(part 1 of 3)
# Autodesk Inventor assembly: 42146-00
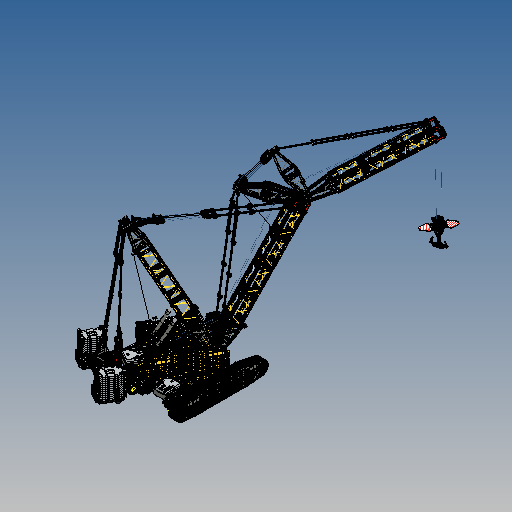
[picture p0: Inventor's stored thumbnail of the model, 512x512]
Saved by Autodesk Inventor 2025 (Build 290162010, 162A)
## iProperties
Created: 2024-11-13
Part Number: 42146-00
Material: Generisch
Document SubType Name: Assembly
Designer: hp.muther
Author: hp.muther
## Documents named in this file (138)
- D:\Inventor\Projekte\LEGO Technik - Raupenkran LR 13000 (42146)\LEGO Technik - Raupenkran LR 13000 (42146).iam
- D:\Inventor\Projekte\LEGO Technik - Raupenkran LR 13000 (42146)\LEGO Technik - Raupenkran LR 13000 (42146)\42146-01.iam
- D:\Inventor\Projekte\LEGO Technik - Raupenkran LR 13000 (42146)\LEGO Technik - Raupenkran LR 13000 (42146)\42146-02.iam
- D:\Inventor\Projekte\LEGO Technik - Raupenkran LR 13000 (42146)\LEGO Technik - Raupenkran LR 13000 (42146)\42146-03.iam
- D:\Inventor\Projekte\LEGO Technik - Raupenkran LR 13000 (42146)\LEGO Pieces\32054-LtBluishGray.ipt
- D:\Inventor\Projekte\LEGO Technik - Raupenkran LR 13000 (42146)\LEGO Pieces\43093-Blue.ipt
- D:\Inventor\Projekte\LEGO Technik - Raupenkran LR 13000 (42146)\LEGO Technik - Raupenkran LR 13000 (42146)\42146-04.iam
- D:\Inventor\Projekte\LEGO Technik - Raupenkran LR 13000 (42146)\LEGO Technik - Raupenkran LR 13000 (42146)\42146-05.iam
- D:\Inventor\Projekte\LEGO Technik - Raupenkran LR 13000 (42146)\LEGO Pieces\6558-Blue.ipt
- D:\Inventor\Projekte\LEGO Technik - Raupenkran LR 13000 (42146)\LEGO Pieces\11214-Red.ipt
- D:\Inventor\Projekte\LEGO Technik - Raupenkran LR 13000 (42146)\LEGO Pieces\73507-Black.ipt
- D:\Inventor\Projekte\LEGO Technik - Raupenkran LR 13000 (42146)\LEGO Pieces\32524-Yellow.ipt
- D:\Inventor\Projekte\LEGO Technik - Raupenkran LR 13000 (42146)\LEGO Technik - Raupenkran LR 13000 (42146)\42146-06.iam
- D:\Inventor\Projekte\LEGO Technik - Raupenkran LR 13000 (42146)\LEGO Technik - Raupenkran LR 13000 (42146)\42146-07.iam
- D:\Inventor\Projekte\LEGO Technik - Raupenkran LR 13000 (42146)\LEGO Technik - Raupenkran LR 13000 (42146)\42146-08.iam
- D:\Inventor\Projekte\LEGO Technik - Raupenkran LR 13000 (42146)\LEGO Pieces\32278-Yellow.ipt
- D:\Inventor\Projekte\LEGO Technik - Raupenkran LR 13000 (42146)\LEGO Pieces\32525-Red.ipt
- D:\Inventor\Projekte\LEGO Technik - Raupenkran LR 13000 (42146)\LEGO Pieces\2780-Black.ipt
- D:\Inventor\Projekte\LEGO Technik - Raupenkran LR 13000 (42146)\LEGO Pieces\24316-ReddishBrown.ipt
- D:\Inventor\Projekte\LEGO Technik - Raupenkran LR 13000 (42146)\LEGO Pieces\46372-LtBluishGray.ipt
- D:\Inventor\Projekte\LEGO Technik - Raupenkran LR 13000 (42146)\LEGO Pieces\15458-DkBluishGray.ipt
- D:\Inventor\Projekte\LEGO Technik - Raupenkran LR 13000 (42146)\LEGO Pieces\67491-Yellow.ipt
- D:\Inventor\Projekte\LEGO Technik - Raupenkran LR 13000 (42146)\LEGO Pieces\40490-LtBluishGray.ipt
- D:\Inventor\Projekte\LEGO Technik - Raupenkran LR 13000 (42146)\LEGO Pieces\39790-Black.ipt
- D:\Inventor\Projekte\LEGO Technik - Raupenkran LR 13000 (42146)\LEGO Pieces\18651-Black.ipt
- D:\Inventor\Projekte\LEGO Technik - Raupenkran LR 13000 (42146)\LEGO Pieces\18654-DkBluishGray.ipt
- D:\Inventor\Projekte\LEGO Technik - Raupenkran LR 13000 (42146)\LEGO Technik - Raupenkran LR 13000 (42146)\42146-09.iam
- D:\Inventor\Projekte\LEGO Technik - Raupenkran LR 13000 (42146)\LEGO Pieces\32140-LtBluishGray.ipt
- D:\Inventor\Projekte\LEGO Technik - Raupenkran LR 13000 (42146)\LEGO Technik - Raupenkran LR 13000 (42146)\42146-10.iam
- D:\Inventor\Projekte\LEGO Technik - Raupenkran LR 13000 (42146)\LEGO Pieces\32278-LtBluishGray.ipt
- D:\Inventor\Projekte\LEGO Technik - Raupenkran LR 13000 (42146)\LEGO Pieces\43857-LtBluishGray.ipt
- D:\Inventor\Projekte\LEGO Technik - Raupenkran LR 13000 (42146)\LEGO Technik - Raupenkran LR 13000 (42146)\42146-11.iam
- D:\Inventor\Projekte\LEGO Technik - Raupenkran LR 13000 (42146)\LEGO Technik - Raupenkran LR 13000 (42146)\42146-12.iam
- D:\Inventor\Projekte\LEGO Technik - Raupenkran LR 13000 (42146)\LEGO Pieces\6629-DkBluishGray.ipt
- D:\Inventor\Projekte\LEGO Technik - Raupenkran LR 13000 (42146)\LEGO Technik - Raupenkran LR 13000 (42146)\42146-13.iam
- D:\Inventor\Projekte\LEGO Technik - Raupenkran LR 13000 (42146)\LEGO Technik - Raupenkran LR 13000 (42146)\42146-14.iam
- D:\Inventor\Projekte\LEGO Technik - Raupenkran LR 13000 (42146)\LEGO Pieces\6589-Tan.ipt
- D:\Inventor\Projekte\LEGO Technik - Raupenkran LR 13000 (42146)\LEGO Pieces\62462-LtBluishGray.ipt
- D:\Inventor\Projekte\LEGO Technik - Raupenkran LR 13000 (42146)\LEGO Pieces\15462-ReddishBrown.ipt
- D:\Inventor\Projekte\LEGO Technik - Raupenkran LR 13000 (42146)\LEGO Pieces\32316-LtBluishGray.ipt
- D:\Inventor\Projekte\LEGO Technik - Raupenkran LR 13000 (42146)\LEGO Pieces\18945-DkBluishGray.ipt
- D:\Inventor\Projekte\LEGO Technik - Raupenkran LR 13000 (42146)\LEGO Pieces\60483-DkBluishGray.ipt
- D:\Inventor\Projekte\LEGO Technik - Raupenkran LR 13000 (42146)\LEGO Pieces\32316-DkBluishGray.ipt
- D:\Inventor\Projekte\LEGO Technik - Raupenkran LR 13000 (42146)\LEGO Pieces\771710-DkBluishGray.ipt
- D:\Inventor\Projekte\LEGO Technik - Raupenkran LR 13000 (42146)\LEGO Pieces\11947-DkBluishGray.ipt
- D:\Inventor\Projekte\LEGO Technik - Raupenkran LR 13000 (42146)\LEGO Pieces\3713-LtBluishGray.ipt
- D:\Inventor\Projekte\LEGO Technik - Raupenkran LR 13000 (42146)\LEGO Technik - Raupenkran LR 13000 (42146)\42146-15.iam
- D:\Inventor\Projekte\LEGO Technik - Raupenkran LR 13000 (42146)\LEGO Pieces\11946-DkBluishGray.ipt
- D:\Inventor\Projekte\LEGO Technik - Raupenkran LR 13000 (42146)\LEGO Technik - Raupenkran LR 13000 (42146)\42146-16.iam
- D:\Inventor\Projekte\LEGO Technik - Raupenkran LR 13000 (42146)\LEGO Technik - Raupenkran LR 13000 (42146)\42146-17.iam
- D:\Inventor\Projekte\LEGO Technik - Raupenkran LR 13000 (42146)\LEGO Pieces\40490-DkBluishGray.ipt
- D:\Inventor\Projekte\LEGO Technik - Raupenkran LR 13000 (42146)\LEGO Technik - Raupenkran LR 13000 (42146)\42146-18.iam
- D:\Inventor\Projekte\LEGO Technik - Raupenkran LR 13000 (42146)\LEGO Technik - Raupenkran LR 13000 (42146)\42146-19.iam
- D:\Inventor\Projekte\LEGO Technik - Raupenkran LR 13000 (42146)\LEGO Technik - Raupenkran LR 13000 (42146)\42146-20.iam
- D:\Inventor\Projekte\LEGO Technik - Raupenkran LR 13000 (42146)\LEGO Pieces\32526-Yellow.ipt
- D:\Inventor\Projekte\LEGO Technik - Raupenkran LR 13000 (42146)\LEGO Pieces\60484-Yellow.ipt
- D:\Inventor\Projekte\LEGO Technik - Raupenkran LR 13000 (42146)\LEGO Pieces\3673-LtBluishGray.ipt
- D:\Inventor\Projekte\LEGO Technik - Raupenkran LR 13000 (42146)\LEGO Technik - Raupenkran LR 13000 (42146)\42146-21.iam
- D:\Inventor\Projekte\LEGO Technik - Raupenkran LR 13000 (42146)\LEGO Pieces\771710-Black.ipt
- D:\Inventor\Projekte\LEGO Technik - Raupenkran LR 13000 (42146)\LEGO Pieces\32002-Tan.ipt
- D:\Inventor\Projekte\LEGO Technik - Raupenkran LR 13000 (42146)\LEGO Pieces\32525-Yellow.ipt
- D:\Inventor\Projekte\LEGO Technik - Raupenkran LR 13000 (42146)\LEGO Pieces\18942-DkBluishGray.ipt
- D:\Inventor\Projekte\LEGO Technik - Raupenkran LR 13000 (42146)\LEGO Pieces\18940-SandBlue.ipt
- D:\Inventor\Projekte\LEGO Technik - Raupenkran LR 13000 (42146)\LEGO Pieces\18654-Black.ipt
- D:\Inventor\Projekte\LEGO Technik - Raupenkran LR 13000 (42146)\LEGO Pieces\32073-LtBluishGray.ipt
- D:\Inventor\Projekte\LEGO Technik - Raupenkran LR 13000 (42146)\LEGO Pieces\60485-LtBluishGray.ipt
- D:\Inventor\Projekte\LEGO Technik - Raupenkran LR 13000 (42146)\LEGO Pieces\32184-LtBluishGray.ipt
- D:\Inventor\Projekte\LEGO Technik - Raupenkran LR 13000 (42146)\LEGO Pieces\77765-MediumStoneGrey.ipt
- D:\Inventor\Projekte\LEGO Technik - Raupenkran LR 13000 (42146)\LEGO Pieces\4265c-Yellow.ipt
- D:\Inventor\Projekte\LEGO Technik - Raupenkran LR 13000 (42146)\LEGO Pieces\32017-DKBluishGray.ipt
- D:\Inventor\Projekte\LEGO Technik - Raupenkran LR 13000 (42146)\LEGO Pieces\6628-Red.ipt
- D:\Inventor\Projekte\LEGO Technik - Raupenkran LR 13000 (42146)\LEGO Technik - Raupenkran LR 13000 (42146)\42146_70902_1.ipt
- D:\Inventor\Projekte\LEGO Technik - Raupenkran LR 13000 (42146)\LEGO Technik - Raupenkran LR 13000 (42146)\42146-22.iam
- D:\Inventor\Projekte\LEGO Technik - Raupenkran LR 13000 (42146)\LEGO Technik - Raupenkran LR 13000 (42146)\42146-23.iam
- D:\Inventor\Projekte\LEGO Technik - Raupenkran LR 13000 (42146)\LEGO Technik - Raupenkran LR 13000 (42146)\42146-24.iam
- D:\Inventor\Projekte\LEGO Technik - Raupenkran LR 13000 (42146)\LEGO Technik - Raupenkran LR 13000 (42146)\42146-25.iam
- D:\Inventor\Projekte\LEGO Technik - Raupenkran LR 13000 (42146)\LEGO Pieces\85824 - HUB.iam
- D:\Inventor\Projekte\LEGO Technik - Raupenkran LR 13000 (42146)\LEGO Pieces\84428-LtBluishGray.ipt
- D:\Inventor\Projekte\LEGO Technik - Raupenkran LR 13000 (42146)\LEGO Pieces\79768-DkBluishGray.ipt
- D:\Inventor\Projekte\LEGO Technik - Raupenkran LR 13000 (42146)\LEGO Pieces\6536-Yellow.ipt
- D:\Inventor\Projekte\LEGO Technik - Raupenkran LR 13000 (42146)\LEGO Pieces\32525-LtBluishGray.ipt
- D:\Inventor\Projekte\LEGO Technik - Raupenkran LR 13000 (42146)\LEGO Technik - Raupenkran LR 13000 (42146)\42146-26.iam
- D:\Inventor\Projekte\LEGO Technik - Raupenkran LR 13000 (42146)\LEGO Pieces\67498-shock absorber.iam
- D:\Inventor\Projekte\LEGO Technik - Raupenkran LR 13000 (42146)\LEGO Technik - Raupenkran LR 13000 (42146)\42146-27.iam
- D:\Inventor\Projekte\LEGO Technik - Raupenkran LR 13000 (42146)\LEGO Pieces\44294-Yellow.ipt
- D:\Inventor\Projekte\LEGO Technik - Raupenkran LR 13000 (42146)\LEGO Pieces\2637-LtBluishGray.ipt
- D:\Inventor\Projekte\LEGO Technik - Raupenkran LR 13000 (42146)\LEGO Pieces\6632-LtBluishGray.ipt
- D:\Inventor\Projekte\LEGO Technik - Raupenkran LR 13000 (42146)\LEGO Pieces\32449-Yellow.ipt
- D:\Inventor\Projekte\LEGO Technik - Raupenkran LR 13000 (42146)\LEGO Pieces\32062-Red.ipt
- D:\Inventor\Projekte\LEGO Technik - Raupenkran LR 13000 (42146)\LEGO Pieces\4519-Yellow.ipt
- D:\Inventor\Projekte\LEGO Technik - Raupenkran LR 13000 (42146)\LEGO Pieces\3707-Black.ipt
- D:\Inventor\Projekte\LEGO Technik - Raupenkran LR 13000 (42146)\LEGO Pieces\32184-Yellow.ipt
- D:\Inventor\Projekte\LEGO Technik - Raupenkran LR 13000 (42146)\LEGO Pieces\48989-LtBluishGray.ipt
- D:\Inventor\Projekte\LEGO Technik - Raupenkran LR 13000 (42146)\LEGO Pieces\32524-LtBluishGray.ipt
- D:\Inventor\Projekte\LEGO Technik - Raupenkran LR 13000 (42146)\LEGO Pieces\40490-Yellow.ipt
- D:\Inventor\Projekte\LEGO Technik - Raupenkran LR 13000 (42146)\LEGO Pieces\18939-LIGHTGREY.ipt
- D:\Inventor\Projekte\LEGO Technik - Raupenkran LR 13000 (42146)\LEGO Technik - Raupenkran LR 13000 (42146)\42146-28.iam
- D:\Inventor\Projekte\LEGO Technik - Raupenkran LR 13000 (42146)\LEGO Technik - Raupenkran LR 13000 (42146)\42146-29.iam
- D:\Inventor\Projekte\LEGO Technik - Raupenkran LR 13000 (42146)\LEGO Pieces\41677-LtBluishGray.ipt
- D:\Inventor\Projekte\LEGO Technik - Raupenkran LR 13000 (42146)\LEGO Pieces\6538c-Red.ipt
- D:\Inventor\Projekte\LEGO Technik - Raupenkran LR 13000 (42146)\LEGO Pieces\11478-LtBluishGray.ipt
- D:\Inventor\Projekte\LEGO Technik - Raupenkran LR 13000 (42146)\LEGO Pieces\42610-LtBluishGray.ipt
- D:\Inventor\Projekte\LEGO Technik - Raupenkran LR 13000 (42146)\LEGO Pieces\26287-LtBluishGray.ipt
- D:\Inventor\Projekte\LEGO Technik - Raupenkran LR 13000 (42146)\LEGO Pieces\92907-LtBluishGray.ipt
- D:\Inventor\Projekte\LEGO Technik - Raupenkran LR 13000 (42146)\LEGO Pieces\80295-White.ipt
- D:\Inventor\Projekte\LEGO Technik - Raupenkran LR 13000 (42146)\LEGO Pieces\23948-Yellow.ipt
- D:\Inventor\Projekte\LEGO Technik - Raupenkran LR 13000 (42146)\LEGO Technik - Raupenkran LR 13000 (42146)\42146-30.iam
- D:\Inventor\Projekte\LEGO Technik - Raupenkran LR 13000 (42146)\LEGO Pieces\4274-Red.ipt
- D:\Inventor\Projekte\LEGO Technik - Raupenkran LR 13000 (42146)\LEGO Pieces\64179-Red.ipt
- D:\Inventor\Projekte\LEGO Technik - Raupenkran LR 13000 (42146)\LEGO Pieces\58176-TransRed.ipt
- D:\Inventor\Projekte\LEGO Technik - Raupenkran LR 13000 (42146)\LEGO Technik - Raupenkran LR 13000 (42146)\42146-31.iam
- D:\Inventor\Projekte\LEGO Technik - Raupenkran LR 13000 (42146)\LEGO Pieces\3706-Red.ipt
- D:\Inventor\Projekte\LEGO Technik - Raupenkran LR 13000 (42146)\LEGO Technik - Raupenkran LR 13000 (42146)\42146-32.iam
- D:\Inventor\Projekte\LEGO Technik - Raupenkran LR 13000 (42146)\LEGO Pieces\62462-Yellow.ipt
- D:\Inventor\Projekte\LEGO Technik - Raupenkran LR 13000 (42146)\LEGO Technik - Raupenkran LR 13000 (42146)\42146-33.iam
- D:\Inventor\Projekte\LEGO Technik - Raupenkran LR 13000 (42146)\LEGO Technik - Raupenkran LR 13000 (42146)\42146-34.iam
- D:\Inventor\Projekte\LEGO Technik - Raupenkran LR 13000 (42146)\LEGO Technik - Raupenkran LR 13000 (42146)\42146-35.iam
- D:\Inventor\Projekte\LEGO Technik - Raupenkran LR 13000 (42146)\LEGO Pieces\4519-LtBluishGray.ipt
- D:\Inventor\Projekte\LEGO Technik - Raupenkran LR 13000 (42146)\LEGO Pieces\41677-DKBluishGray.ipt
- D:\Inventor\Projekte\LEGO Technik - Raupenkran LR 13000 (42146)\LEGO Pieces\25214-LtBluishGray.ipt
- D:\Inventor\Projekte\LEGO Technik - Raupenkran LR 13000 (42146)\LEGO Technik - Raupenkran LR 13000 (42146)\42146-36.iam
- D:\Inventor\Projekte\LEGO Technik - Raupenkran LR 13000 (42146)\LEGO Pieces\4162-LtBluishGray.ipt
- D:\Inventor\Projekte\LEGO Technik - Raupenkran LR 13000 (42146)\LEGO Pieces\3022-Yellow.ipt
- D:\Inventor\Projekte\LEGO Technik - Raupenkran LR 13000 (42146)\LEGO Pieces\3710-Yellow.ipt
- D:\Inventor\Projekte\LEGO Technik - Raupenkran LR 13000 (42146)\LEGO Pieces\2420-Yellow.ipt
- D:\Inventor\Projekte\LEGO Technik - Raupenkran LR 13000 (42146)\LEGO Pieces\3020-Yellow.ipt
- D:\Inventor\Projekte\LEGO Technik - Raupenkran LR 13000 (42146)\LEGO Pieces\44873-LtBluishGray.ipt
- D:\Inventor\Projekte\LEGO Technik - Raupenkran LR 13000 (42146)\LEGO Pieces\87994-LtBluishGray.ipt
- D:\Inventor\Projekte\LEGO Technik - Raupenkran LR 13000 (42146)\LEGO Pieces\63037-LtBluishGray.ipt
- D:\Inventor\Projekte\LEGO Technik - Raupenkran LR 13000 (42146)\LEGO Pieces\63965-LtBluishGray.ipt
- D:\Inventor\Projekte\LEGO Technik - Raupenkran LR 13000 (42146)\LEGO Pieces\4274-LtBluishGray.ipt
- D:\Inventor\Projekte\LEGO Technik - Raupenkran LR 13000 (42146)\LEGO Pieces\3023-Black.ipt
- D:\Inventor\Projekte\LEGO Technik - Raupenkran LR 13000 (42146)\LEGO Pieces\54200-TransClear.ipt
- D:\Inventor\Projekte\LEGO Technik - Raupenkran LR 13000 (42146)\LEGO Pieces\32291-DkBluishGray.ipt
- D:\Inventor\Projekte\LEGO Technik - Raupenkran LR 13000 (42146)\LEGO Technik - Raupenkran LR 13000 (42146)\42146-37.iam
- D:\Inventor\Projekte\LEGO Technik - Raupenkran LR 13000 (42146)\LEGO Technik - Raupenkran LR 13000 (42146)\42146-38.ipt
- D:\Inventor\Projekte\LEGO Technik - Raupenkran LR 13000 (42146)\LEGO Technik - Raupenkran LR 13000 (42146)\42146-39.ipt
- D:\Inventor\Projekte\LEGO Technik - Raupenkran LR 13000 (42146)\LEGO Technik - Raupenkran LR 13000 (42146)\42146-40.ipt
## Components (648 placed, 137 different names)
1. 42146-38:1 — Passend:501, Passend:502, Winkel:20
2. 80295-White:1 — Einfügen:488
3. 23948-Yellow:1 — Einfügen:487, Einfügen:488, Passend:502
4. 42146-39:1 — Passend:503, Passend:504, Winkel:21
5. 80295-White:2 — Einfügen:536
6. 23948-Yellow:2 — Passend:504
7. 42146-40:1 — Passend:505, Passend:506, Winkel:22
8. 80295-White:3 — Einfügen:577
9. 80295-White:4 — Einfügen:576, Einfügen:577
10. 23948-Yellow:3 — Einfügen:576, Einfügen:578, Passend:506
11. 42146-01:1 [sub-assembly] — Passend:1, Passend:2, Passend:3, Fluchtend:1, Einfügen:1, Passend:4, Einfügen:2, Passend:5, Einfügen:5, Einfügen:6, Passend:10, Passend:11, Passend:12, Einfügen:15, Einfügen:16, Einfügen:17, Einfügen:18, Passend:13, Einfügen:20, Einfügen:21, Einfügen:22, Einfügen:23, Einfügen:24, Einfügen:25, Einfügen:26, Einfügen:27, Einfügen:28
12. 42146-02:1 [sub-assembly] — Einfügen:1, Passend:4, Einfügen:4, Einfügen:7, Einfügen:8, Einfügen:71, Passend:42, Einfügen:74
13. 42146-03:1 [sub-assembly] — Einfügen:2, Passend:5, Einfügen:3, Passend:6, Passend:7, Einfügen:72, Passend:41, Winkel:19
14. 42146-04:1 [sub-assembly] — Einfügen:7, Passend:6
15. 42146-05:1 [sub-assembly] — Einfügen:8, Passend:7, Passend:14, Einfügen:19
16. 42146-06:1 [sub-assembly] — Passend:13, Passend:14
17. 42146-07:1 [sub-assembly] — Einfügen:19, Passend:32, Passend:34, Einfügen:33, Passend:36, Passend:17, Passend:18, Passend:19, Passend:20, Drehung:1, Drehung:2, Passend:25, Passend:33, Passend:35, Passend:37, Passend:38
18. 42146-08:1 - beweglich [sub-assembly] — Einfügen:28, Passend:15, Einfügen:45, Passend:22, Einfügen:46, Passend:23, Einfügen:47
19. 42146-09:1 [sub-assembly] — Einfügen:76, Passend:43, Einfügen:80, Passend:44, Einfügen:86, Einfügen:87, Passend:49, Einfügen:94, Einfügen:96, Einfügen:98, Einfügen:100, Einfügen:101, Einfügen:106, Passend:52, Einfügen:121, Passend:59, Einfügen:130, Einfügen:146, Passend:67, Einfügen:181, Passend:82, Einfügen:183, Passend:84, Einfügen:195, Einfügen:196, Einfügen:197, Einfügen:198, Einfügen:207, Einfügen:208
20. 42146-10:1 [sub-assembly] — Einfügen:81, Passend:45, Einfügen:85, Passend:46, Passend:47, Einfügen:88, Einfügen:92, Einfügen:93, Einfügen:95, Einfügen:97, Einfügen:99, Einfügen:113, Passend:56, Einfügen:151, Passend:71, Passend:80, Einfügen:180, Passend:81, Einfügen:182, Passend:83, Einfügen:184, Passend:85, Einfügen:199, Einfügen:200, Einfügen:201, Einfügen:202, Einfügen:205, Einfügen:206
21. 42146-11:1 [sub-assembly] — Einfügen:101, Passend:50, Einfügen:102, Einfügen:103, Einfügen:104, Einfügen:105
22. 42146-12:1 [sub-assembly] — Einfügen:106, Passend:52, Einfügen:111, Passend:54, Einfügen:112, Passend:55, Einfügen:192, Passend:89, Passend:93
23. 42146-13:1 [sub-assembly] — Einfügen:113, Passend:56, Einfügen:118, Passend:58, Einfügen:119, Einfügen:120, Einfügen:188, Passend:87, Passend:90, Passend:95
24. 42146-14:1 [sub-assembly] — Einfügen:121, Passend:59, Passend:61, Passend:68
25. 42146-15:1 [sub-assembly] — Einfügen:151, Passend:71, Einfügen:179, Einfügen:209, Passend:94
26. 42146-16:1 [sub-assembly] — Einfügen:182, Passend:83
27. 42146-16:2 [sub-assembly] — Einfügen:181, Passend:82
28. 42146-17:1 [sub-assembly] — Einfügen:183, Passend:84
29. 42146-17:2 [sub-assembly] — Einfügen:184, Passend:85
30. 42146-18:1 [sub-assembly] — Einfügen:209, Passend:94
31. 42146-19:1 [sub-assembly] — Passend:95, Passend:96, Winkel:1
32. 42146-19:2 [sub-assembly] — Passend:97, Winkel:2, Passend:98
33. 42146-20:1 [sub-assembly] — Einfügen:210, Passend:99, Einfügen:211, Einfügen:212, Einfügen:213, Einfügen:214, Einfügen:215, Einfügen:216, Einfügen:217, Einfügen:218, Einfügen:219, Einfügen:220, Einfügen:221, Einfügen:226, Einfügen:227, Einfügen:228, Einfügen:229, Einfügen:230, Einfügen:231, Einfügen:232, Einfügen:233, Einfügen:234, Einfügen:235, Einfügen:236, Einfügen:237, Einfügen:238, Einfügen:243, Einfügen:244, Einfügen:252, Passend:104, Einfügen:251, Passend:105, Einfügen:259, Einfügen:260, Passend:106, Passend:107, Einfügen:296, Einfügen:297, Einfügen:350, Passend:154, Einfügen:352, Einfügen:353, Einfügen:366, Einfügen:367, Einfügen:386, Einfügen:387, Einfügen:388, Einfügen:443, Einfügen:444, Einfügen:536, Passend:501, Winkel:20, Passend:503, Winkel:21, Passend:505, Winkel:22
34. 42146-21:1 [sub-assembly] — Einfügen:279, Passend:114, Passend:115, Passend:116, Passend:117, Passend:118, Einfügen:316, Passend:148, Passend:149
35. 42146-22:1 [sub-assembly] — Passend:145, Passend:146, Passend:147, Einfügen:381, Passend:239, Einfügen:382, Einfügen:383, Einfügen:384, Einfügen:385, Passend:240
36. 42146-23:1 [sub-assembly] — Einfügen:324, Passend:148, Passend:152, Passend:153, Passend:232, Passend:233, Passend:234
37. 42146-24:1 [sub-assembly] — Einfügen:323, Passend:149, Passend:150, Passend:151, Passend:163, Passend:164, Passend:165
38. 42146-25:1 [sub-assembly] — Einfügen:354, Passend:155, Passend:156, Passend:157, Einfügen:370, Passend:158, Einfügen:371, Passend:161, Einfügen:487, Einfügen:544, Passend:452, Einfügen:578
39. 42146-26:1 [sub-assembly] — Einfügen:388, Passend:243, Passend:244, Einfügen:395, Passend:245
40. 67498-shock absorber:1 [sub-assembly] — Einfügen:391, Einfügen:392, Einfügen:394, Passend:244
41. 67498-shock absorber:2 [sub-assembly] — Einfügen:389, Einfügen:390, Einfügen:393, Passend:243
42. 42146-27:1 [sub-assembly] — Einfügen:395, Passend:245, Einfügen:396, Einfügen:397, Einfügen:412, Passend:423, Fluchtend:14, Passend:435
43. 42146-28:1 [sub-assembly] — Einfügen:445, Passend:426, Einfügen:452, Passend:429, Einfügen:490, Passend:440, Passend:448, Einfügen:574, Einfügen:575, Passend:497
44. 42146-29:1 [sub-assembly] — Einfügen:452, Passend:429, Einfügen:485, Einfügen:486
45. 42146-30:1 [sub-assembly] — Winkel:14, Passend:498, Passend:500
46. 42146-31:1 [sub-assembly] — Winkel:14
47. 42146-32:1 [sub-assembly] — Einfügen:490, Passend:440, Passend:448
48. 42146-33:1 [sub-assembly] — Einfügen:542, Passend:450
49. 42146-34:1 [sub-assembly] — Einfügen:543, Passend:451, Einfügen:557, Passend:455, Passend:471, Passend:475, Passend:476, Passend:477, Einfügen:563, Einfügen:573, Winkel:18
50. 42146-35:1 [sub-assembly] — Einfügen:544, Passend:452
51. 42146-36:1 [sub-assembly] — Einfügen:552, Passend:454, Passend:473, Passend:474, Fluchtend:32
52. 42146-37:1 [sub-assembly] — Passend:498, Passend:499, Passend:500, Winkel:23
53. 84428-LtBluishGray:1 — Passend:163, Passend:164, Passend:165, Passend:166, Passend:167, Passend:168
54. 84428-LtBluishGray:2 — Passend:166, Passend:167, Passend:168, Passend:172, Passend:173, Passend:174
55. 84428-LtBluishGray:3 — Passend:172, Passend:173, Passend:174
56. 84428-LtBluishGray:4 — Passend:196, Passend:197, Passend:198
57. 84428-LtBluishGray:5 — Passend:193, Passend:194, Passend:195
58. 84428-LtBluishGray:6
59. 84428-LtBluishGray:7
60. 84428-LtBluishGray:8
61. 84428-LtBluishGray:9 — Passend:196, Passend:197, Passend:198
62. 84428-LtBluishGray:10
63. 84428-LtBluishGray:11
64. 84428-LtBluishGray:12 — Passend:193, Passend:194, Passend:195
65. 84428-LtBluishGray:13 — Passend:232, Passend:233, Passend:234
66. 84428-LtBluishGray:14
67. 84428-LtBluishGray:15
68. 84428-LtBluishGray:16
69. 84428-LtBluishGray:17
70. 84428-LtBluishGray:18
71. 84428-LtBluishGray:19
72. 84428-LtBluishGray:20
73. 84428-LtBluishGray:21
74. 84428-LtBluishGray:22
75. 84428-LtBluishGray:23
76. 84428-LtBluishGray:24
77. 32054-LtBluishGray:1 — Einfügen:3
78. 32054-LtBluishGray:2 — Einfügen:4
79. 43093-Blue:1 — Einfügen:5
80. 43093-Blue:2 — Einfügen:6
81. 6558-Blue:1 — Einfügen:14, Passend:21
82. 6558-Blue:2 — Einfügen:10, Passend:8, Passend:9
83. 11214-Red:1 — Einfügen:18
84. 11214-Red:2 — Einfügen:17
85. 11214-Red:3 — Einfügen:16
86. 11214-Red:4 — Einfügen:15
87. 6558-Blue:3 — Einfügen:9, Einfügen:11
88. 6558-Blue:4 — Einfügen:13, Einfügen:40
89. 73507-Black:1 — Einfügen:12, Passend:8, Einfügen:14
90. 73507-Black:2 — Einfügen:11, Passend:9, Passend:11, Passend:12, Passend:10, Einfügen:13
91. 32524-Yellow:1 — Einfügen:9, Einfügen:10, Einfügen:12
92. 32054-LtBluishGray:3 — Einfügen:25
93. 32054-LtBluishGray:4 — Einfügen:26
94. 32054-LtBluishGray:5 — Einfügen:27
95. 32054-LtBluishGray:6 — Einfügen:24
96. 32054-LtBluishGray:7 — Einfügen:20
97. 32054-LtBluishGray:8 — Einfügen:21, Passend:15
98. 32054-LtBluishGray:9 — Einfügen:22
99. 32054-LtBluishGray:10 — Einfügen:23
100. 32278-Yellow:1 — Einfügen:38, Einfügen:39, Einfügen:40, Passend:21
101. 24316-ReddishBrown:1 — Einfügen:36, Einfügen:39
102. 46372-LtBluishGray:1 — Einfügen:36, Drehung:2
103. 24316-ReddishBrown:2 — Einfügen:37, Einfügen:38
104. 46372-LtBluishGray:2 — Einfügen:37, Drehung:1
105. 32278-Yellow:5 — Passend:32, Passend:18, Passend:33, Winkel:19
106. 32278-Yellow:2 — Passend:36, Passend:17, Passend:37
107. 32278-Yellow:3 — Einfügen:33, Passend:20
108. 32278-Yellow:4 — Passend:34, Einfügen:35, Passend:16, Passend:19, Einfügen:57, Passend:35, Einfügen:58
109. 32525-Red:1 — Einfügen:29, Einfügen:30, Einfügen:60, Passend:40
110. 2780-Black:1 — Einfügen:29, Einfügen:35
111. 2780-Black:2 — Einfügen:30, Passend:16
112. 15458-DkBluishGray:1 — Einfügen:41, Einfügen:42, Einfügen:46, Einfügen:52, Einfügen:53, Einfügen:56, Einfügen:59
113. 15458-DkBluishGray:2 — Einfügen:47, Passend:24, Einfügen:50, Einfügen:51, Einfügen:55
114. 6558-Blue:5 — Einfügen:42
115. 6558-Blue:6 — Einfügen:41, Passend:23, Passend:24
116. 15458-DkBluishGray:3 — Einfügen:45, Einfügen:48, Einfügen:49, Einfügen:54
117. 6558-Blue:7
118. 6558-Blue:8 — Passend:22
119. 2780-Black:3 — Einfügen:52
120. 2780-Black:4 — Einfügen:48
121. 2780-Black:5 — Einfügen:49, Passend:39
122. 2780-Black:6 — Einfügen:50
123. 2780-Black:7 — Einfügen:53
124. 2780-Black:8 — Einfügen:51
125. 2780-Black:9 — Einfügen:56, Passend:51
126. 2780-Black:10 — Einfügen:55
127. 2780-Black:11 — Einfügen:54
128. 67491-Yellow:1 — Einfügen:57, Passend:25, Einfügen:210, Passend:99
129. 67491-Yellow:2 — Einfügen:58, Passend:38
130. 40490-LtBluishGray:1 — Einfügen:59, Passend:39, Passend:499
131. 32054-LtBluishGray:11 — Einfügen:61
132. 32054-LtBluishGray:12 — Einfügen:62
133. 39790-Black:1 — Einfügen:60, Passend:40, Einfügen:61, Einfügen:62, Passend:51
134. 67491-Yellow:3 — Einfügen:63, Einfügen:64, Einfügen:65, Einfügen:66, Einfügen:72, Passend:41, Einfügen:81
135. 6558-Blue:9 — Einfügen:63, Passend:45
136. 6558-Blue:10 — Einfügen:65
137. 6558-Blue:11 — Einfügen:66
138. 6558-Blue:12 — Einfügen:64
139. 67491-Yellow:4 — Einfügen:71, Passend:42, Einfügen:73, Einfügen:75, Einfügen:76, Passend:43
140. 6558-Blue:13
141. 6558-Blue:14
142. 6558-Blue:15
143. 6558-Blue:16
144. 18651-Black:1 — Einfügen:74, Passend:48
145. 6558-Blue:17 — Einfügen:73
146. 18654-DkBluishGray:1 — Einfügen:75, Einfügen:89
147. 32140-LtBluishGray:1 — Einfügen:77, Einfügen:78, Einfügen:79, Einfügen:80
148. 6558-Blue:18 — Einfügen:78, Passend:44
149. 6558-Blue:19 — Einfügen:77
150. 2780-Black:12 — Einfügen:79
151. 32140-LtBluishGray:2 — Einfügen:82, Einfügen:83, Einfügen:84, Einfügen:85
152. 6558-Blue:20 — Einfügen:83, Passend:46
153. 6558-Blue:21 — Einfügen:82
154. 2780-Black:13 — Einfügen:84
155. 32278-LtBluishGray:1 — Einfügen:86, Passend:47
156. 32054-LtBluishGray:13 — Einfügen:88
157. 32054-LtBluishGray:14 — Einfügen:87
158. 43857-LtBluishGray:1 — Einfügen:89, Passend:48
159. 32278-Yellow:6 — Einfügen:90, Einfügen:91, Einfügen:92
160. 2780-Black:14 — Einfügen:90
161. 2780-Black:15 — Einfügen:91, Passend:49
162. 32054-LtBluishGray:15 — Einfügen:95
163. 32054-LtBluishGray:16 — Einfügen:96
164. 6558-Blue:22 — Einfügen:98
165. 6558-Blue:23 — Einfügen:97, Passend:50
166. 6558-Blue:24 — Einfügen:99
167. 6558-Blue:25 — Einfügen:100
168. 11214-Red:5 — Einfügen:93
169. 11214-Red:6 — Einfügen:94
170. 32054-LtBluishGray:17 — Einfügen:104
171. 32054-LtBluishGray:18 — Einfügen:103
172. 32054-LtBluishGray:19 — Einfügen:102
173. 32054-LtBluishGray:20 — Einfügen:105
174. 2780-Black:16 — Einfügen:108, Passend:54
175. 2780-Black:17 — Einfügen:107
176. 43093-Blue:3 — Einfügen:110, Passend:53
177. 43093-Blue:4 — Einfügen:109
178. 32524-Yellow:2 — Einfügen:107, Einfügen:112, Passend:55
179. 6629-DkBluishGray:1 — Einfügen:108, Einfügen:109, Einfügen:110, Passend:53, Einfügen:111
180. 2780-Black:18 — Einfügen:115
181. 2780-Black:19
182. 43093-Blue:5 — Einfügen:117
183. 43093-Blue:6 — Einfügen:116, Einfügen:120
184. 32524-Yellow:3 — Einfügen:118, Passend:58
185. 6629-DkBluishGray:2 — Einfügen:115, Einfügen:116, Einfügen:117, Einfügen:119
186. 6589-Tan:1 — Einfügen:124, Einfügen:125
187. 6589-Tan:2 — Einfügen:126
188. 62462-LtBluishGray:1 — Einfügen:125, Einfügen:126
189. 2780-Black:20 — Einfügen:127
190. 6558-Blue:26 — Einfügen:122
191. 6558-Blue:27 — Einfügen:123, Passend:60, Passend:61
192. 15462-ReddishBrown:1 — Einfügen:124, Einfügen:129
193. 32316-LtBluishGray:1 — Einfügen:128, Passend:60, Einfügen:129
194. 32316-LtBluishGray:2 — Einfügen:122, Einfügen:123, Einfügen:127, Einfügen:128, Einfügen:130
195. 2780-Black:21 — Einfügen:132, Passend:62
196. 2780-Black:22 — Einfügen:134, Passend:63
197. 6558-Blue:28 — Einfügen:137
198. 11214-Red:7 — Einfügen:131
199. 2780-Black:23 — Einfügen:136, Passend:64
200. 6558-Blue:29 — Einfügen:143
201. 2780-Black:24 — Einfügen:144, Passend:66
202. 18945-DkBluishGray:1 — Einfügen:135, Passend:63, Einfügen:136, Einfügen:137, Einfügen:138, Einfügen:150, Passend:70, Einfügen:193, Einfügen:194, Passend:98
203. 60483-DkBluishGray:1 — Einfügen:131, Einfügen:132, Einfügen:133
204. 32316-DkBluishGray:1 — Einfügen:133, Einfügen:134, Einfügen:135, Passend:62
205. 771710-DkBluishGray:1 — Einfügen:138, Passend:64, Einfügen:140, Einfügen:141, Einfügen:142, Passend:65, Einfügen:146, Passend:67, Winkel:2
206. 32316-DkBluishGray:2 — Einfügen:142, Passend:65, Einfügen:145, Passend:66
207. 11947-DkBluishGray:1 — Einfügen:143, Einfügen:144, Einfügen:145
208. 24316-ReddishBrown:3 — Einfügen:139, Einfügen:140, Passend:68, Passend:97
209. 3713-LtBluishGray:1 — Einfügen:139
210. 2780-Black:25 — Einfügen:141
211. 2780-Black:26 — Passend:70
212. 43093-Blue:7
213. 43093-Blue:8
214. 6629-DkBluishGray:3 — Einfügen:150
215. 6589-Tan:3
216. 6589-Tan:4
217. 62462-LtBluishGray:2
218. 2780-Black:27
219. 6558-Blue:30 — Passend:80
220. 6558-Blue:31
221. 15462-ReddishBrown:2
222. 32316-LtBluishGray:3 — Einfügen:179
223. 32316-LtBluishGray:4
224. 2780-Black:28
225. 2780-Black:29
226. 6558-Blue:32
227. 11214-Red:8
228. 2780-Black:30
229. 6558-Blue:33 — Einfügen:172
230. 2780-Black:31 — Einfügen:173
231. 18945-DkBluishGray:2 — Einfügen:178, Passend:79, Einfügen:203, Einfügen:204
232. 60483-DkBluishGray:2
233. 32316-DkBluishGray:3
234. 771710-DkBluishGray:2 — Einfügen:169, Einfügen:180, Passend:81, Winkel:1
235. 32316-DkBluishGray:4 — Einfügen:174
236. 11946-DkBluishGray:1 — Einfügen:172, Einfügen:173, Einfügen:174
237. 24316-ReddishBrown:4 — Einfügen:169, Passend:96
238. 3713-LtBluishGray:2
239. 2780-Black:32
240. 2780-Black:33 — Einfügen:175, Passend:79
241. 43093-Blue:9 — Einfügen:177
242. 43093-Blue:10 — Einfügen:176
243. 6629-DkBluishGray:4 — Einfügen:175, Einfügen:176, Einfügen:177, Einfügen:178
244. 2780-Black:34 — Passend:87
245. 43093-Blue:11
246. 43093-Blue:12
247. 6629-DkBluishGray:5 — Einfügen:188
248. 2780-Black:35 — Passend:89
249. 43093-Blue:13
250. 43093-Blue:14
251. 6629-DkBluishGray:6 — Einfügen:192
252. 2780-Black:36 — Einfügen:195
253. 2780-Black:37 — Einfügen:196
254. 2780-Black:38 — Einfügen:194
255. 2780-Black:39 — Einfügen:193, Passend:92
256. 2780-Black:40 — Einfügen:198
257. 2780-Black:41 — Einfügen:197
258. 2780-Black:42 — Einfügen:201
259. 2780-Black:43 — Einfügen:202
260. 2780-Black:44 — Einfügen:203
261. 2780-Black:45 — Einfügen:204, Passend:91
262. 2780-Black:46 — Einfügen:199
263. 2780-Black:47 — Einfügen:200
264. 40490-DkBluishGray:1 — Einfügen:205, Passend:91
265. 40490-DkBluishGray:2 — Einfügen:206, Passend:90
266. 40490-DkBluishGray:3 — Einfügen:208, Passend:93
267. 40490-DkBluishGray:4 — Einfügen:207, Passend:92
268. 2780-Black:64 — Einfügen:254
269. 2780-Black:65 — Einfügen:255, Passend:106
270. 60484-Yellow:1 — Einfügen:253, Einfügen:254, Einfügen:255, Einfügen:260, Einfügen:288
271. 3673-LtBluishGray:1 — Einfügen:253
272. 2780-Black:66 — Passend:107
273. 2780-Black:67
274. 60484-Yellow:2 — Einfügen:259, Einfügen:289
275. 3673-LtBluishGray:2
276. 67491-Yellow:7 — Einfügen:263, Einfügen:264, Einfügen:269, Einfügen:270, Einfügen:271, Einfügen:272, Passend:108, Einfügen:298, Einfügen:318
277. 2780-Black:68 — Passend:144
278. 2780-Black:69
279. 2780-Black:70 — Einfügen:263
280. 2780-Black:71 — Einfügen:264
281. 2780-Black:72 — Einfügen:274
282. 6558-Blue:50 — Einfügen:270
283. 6558-Blue:51 — Einfügen:271
284. 2780-Black:73 — Einfügen:269
285. 67491-Yellow:8 — Einfügen:273, Einfügen:274, Einfügen:279, Passend:114, Passend:145, Passend:146, Einfügen:319, Einfügen:320, Einfügen:323, Einfügen:335, Einfügen:336
286. 2780-Black:74 — Passend:109
287. 2780-Black:75
288. 2780-Black:76
289. 2780-Black:77
290. 67491-Yellow:9 — Einfügen:273, Passend:109, Einfügen:275, Einfügen:276, Einfügen:277, Passend:111, Einfügen:278, Passend:113, Einfügen:299
291. 67491-Yellow:10 — Passend:110, Passend:111, Passend:112
292. 2780-Black:78 — Einfügen:275
293. 6558-Blue:52 — Einfügen:277, Passend:110
294. 6558-Blue:53 — Einfügen:276, Passend:112
295. 32526-Yellow:1 — Einfügen:245, Einfügen:248, Einfügen:249, Einfügen:251
296. 32526-Yellow:2 — Einfügen:246, Einfügen:247, Einfügen:250, Einfügen:252
297. 2780-Black:62 — Einfügen:245
298. 2780-Black:63 — Einfügen:246
299. 6558-Blue:46 — Einfügen:249, Passend:105
300. 6558-Blue:47 — Einfügen:247
301. 6558-Blue:48 — Einfügen:248, Passend:108
302. 6558-Blue:49 — Einfügen:250, Passend:104
303. 2780-Black:48 — Einfügen:218, Passend:101
304. 2780-Black:49 — Einfügen:219
305. 2780-Black:50 — Einfügen:221
306. 2780-Black:51 — Einfügen:220
307. 6558-Blue:34 — Einfügen:211
308. 6558-Blue:35 — Einfügen:214, Passend:100
309. 6558-Blue:36 — Einfügen:215
310. 6558-Blue:37 — Einfügen:212
311. 6558-Blue:38 — Einfügen:213
312. 11214-Red:9 — Einfügen:217
313. 11214-Red:10 — Einfügen:216
314. 67491-Yellow:5 — Einfügen:222, Einfügen:223, Einfügen:224, Einfügen:225, Einfügen:226, Passend:100, Einfügen:272
315. 40490-LtBluishGray:2 — Einfügen:227, Passend:101, Einfügen:542, Passend:450
316. 2780-Black:52 — Einfügen:223
317. 2780-Black:53 — Einfügen:225
318. 2780-Black:54 — Einfügen:224
319. 6558-Blue:39 — Einfügen:222
320. 2780-Black:55 — Einfügen:236, Passend:102
321. 2780-Black:56 — Einfügen:230
322. 2780-Black:57 — Einfügen:237
323. 2780-Black:58 — Einfügen:238
324. 6558-Blue:40 — Einfügen:228
325. 6558-Blue:41 — Einfügen:234, Passend:103
326. 6558-Blue:42 — Einfügen:235
327. 6558-Blue:43 — Einfügen:229
328. 6558-Blue:44 — Einfügen:233
329. 11214-Red:11 — Einfügen:231
330. 11214-Red:12 — Einfügen:232
331. 67491-Yellow:6 — Einfügen:239, Einfügen:240, Einfügen:241, Einfügen:242, Einfügen:244, Passend:103, Einfügen:278
332. 2780-Black:59 — Einfügen:240, Passend:113
333. 2780-Black:60 — Einfügen:242
334. 2780-Black:61 — Einfügen:241
335. 6558-Blue:45 — Einfügen:239
336. 40490-LtBluishGray:3 — Einfügen:243, Passend:102, Einfügen:543, Passend:451
337. 32054-LtBluishGray:21 — Einfügen:293, Passend:115
338. 2780-Black:81 — Einfügen:292
339. 32278-Yellow:7 — Einfügen:292, Einfügen:293, Einfügen:296
340. 32054-LtBluishGray:22 — Passend:116
341. 2780-Black:82
342. 32278-Yellow:8 — Einfügen:297
343. 32525-Yellow:1 — Einfügen:298, Passend:118
344. 32525-Yellow:2 — Einfügen:299, Passend:117
345. 18942-DkBluishGray:1 — Passend:119, Passend:120, Passend:121, Passend:122, Passend:129, Passend:130, Einfügen:411, Fluchtend:8
346. 18940-SandBlue:1 — Passend:119, Passend:120, Passend:124, Passend:126, Passend:127, Passend:128, Passend:131, Einfügen:315, Passend:136, Einfügen:316
347. 18654-Black:1 — Passend:125, Passend:126
348. 32073-LtBluishGray:1 — Einfügen:300, Passend:129, Passend:133, Passend:127
349. 60485-LtBluishGray:1 — Einfügen:301, Passend:130, Passend:132
350. 32184-LtBluishGray:1 — Einfügen:300, Einfügen:301, Passend:131, Einfügen:302, Fluchtend:2, Einfügen:307, Passend:134
351. 77765-MediumStoneGrey:1 — Passend:121, Passend:123, Passend:134
352. 77765-MediumStoneGrey:2 — Passend:122, Passend:124, Passend:125, Passend:128
353. 4265c-Yellow:1 — Einfügen:302, Fluchtend:2, Einfügen:304, Einfügen:308
354. 32184-LtBluishGray:2 — Passend:132, Passend:133, Einfügen:306, Passend:123
355. 4265c-Yellow:2 — Einfügen:305, Einfügen:309
356. 4265c-Yellow:3 — Einfügen:305
357. 4265c-Yellow:4 — Einfügen:304
358. 32017-DKBluishGray:1 — Einfügen:308, Passend:137
359. 32017-DKBluishGray:2 — Einfügen:309, Passend:138
360. 6628-Red:1 — Einfügen:306
361. 6628-Red:2 — Einfügen:307
362. 32073-LtBluishGray:2 — Einfügen:312, Einfügen:314, Passend:136
363. 3713-LtBluishGray:3 — Einfügen:310, Einfügen:312, Passend:139, Passend:142
364. 6558-Blue:54 — Einfügen:311, Passend:135
365. 60483-DkBluishGray:3 — Einfügen:310, Einfügen:311, Einfügen:315
366. 3713-LtBluishGray:4 — Einfügen:314, Passend:140, Passend:141
367. 60483-DkBluishGray:4 — Passend:135, Winkel:3
368. 42146_70902_1:1 — Passend:140, Passend:141, Passend:143, Winkel:3
369. 42146_70902_1:2 — Passend:139, Passend:142, Passend:143
370. 2780-Black:83 — Einfügen:317
371. 67491-Yellow:11 — Einfügen:317, Einfügen:318, Passend:144, Passend:147, Einfügen:321, Einfügen:322, Einfügen:324, Einfügen:333, Einfügen:334
372. 771710-Black:1 — Einfügen:280, Einfügen:281, Einfügen:282, Einfügen:286, Einfügen:289, Einfügen:290, Einfügen:372
373. 43093-Blue:15 — Einfügen:280, Passend:162
374. 43093-Blue:16 — Einfügen:281
375. 2780-Black:79 — Einfügen:282
376. 32002-Tan:1 — Einfügen:287, Passend:137
377. 32002-Tan:2 — Einfügen:286, Passend:138
378. 771710-Black:2 — Einfügen:283, Einfügen:284, Einfügen:287, Einfügen:288, Einfügen:291
379. 43093-Blue:17 — Einfügen:283
380. 43093-Blue:18 — Einfügen:284
381. 2780-Black:80
382. 40490-LtBluishGray:4 — Einfügen:290, Einfügen:291
383. 77765-MediumStoneGrey:3 — Einfügen:322
384. 77765-MediumStoneGrey:4 — Einfügen:321
385. 77765-MediumStoneGrey:5 — Einfügen:320
386. 77765-MediumStoneGrey:6 — Einfügen:319
387. 43857-LtBluishGray:2 — Einfügen:325, Einfügen:326, Einfügen:335
388. 2780-Black:84 — Einfügen:326
389. 2780-Black:85 — Einfügen:325, Passend:151
390. 43857-LtBluishGray:3 — Einfügen:336
391. 2780-Black:86
392. 2780-Black:87 — Passend:150
393. 43857-LtBluishGray:4 — Einfügen:334
394. 2780-Black:88
395. 2780-Black:89 — Passend:153
396. 43857-LtBluishGray:5 — Einfügen:333
397. 2780-Black:90
398. 2780-Black:91 — Passend:152
399. 2780-Black:92
400. 67491-Yellow:12 — Einfügen:338, Einfügen:339, Einfügen:340, Einfügen:341, Einfügen:342, Einfügen:343, Einfügen:344, Einfügen:345, Einfügen:346, Einfügen:347, Einfügen:348, Einfügen:349, Einfügen:350, Einfügen:354, Einfügen:368, Einfügen:369
401. 2780-Black:93 — Einfügen:338
402. 2780-Black:94 — Einfügen:339
403. 2780-Black:95 — Einfügen:340
404. 2780-Black:96 — Einfügen:341
405. 2780-Black:97 — Einfügen:342, Passend:155
406. 2780-Black:98 — Einfügen:344
407. 2780-Black:99 — Einfügen:343